# Autodesk Inventor assembly: LHSA 14
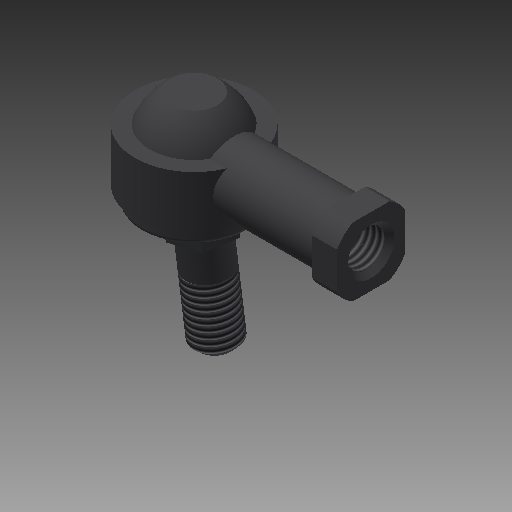
[picture p0: Inventor's stored thumbnail of the model, 512x512]
Saved by Autodesk Inventor 2018 (Build 220112000, 112)
## iProperties
Category: PARTsolutions
Company: IKO
Created: 2017-09-07
Part Number: LHSA 14
Catalog Web Link: www.cadenas.de
Description: LHSA-
Vendor: IKO
Document SubType Name: Assembly
Designer: psAdmin
Manufacturer: IKO
PSOL_IDENT_0: {$CADENAS_DATA\23d-libs\iko\iko_bearings\l_balls\lhsa_1_asmtab.prj},159 {VTYP=3D},{STYP=ASSTAB},{NB=
PSOL_IDENT_1: LHSA 14},{LINA=LHSA 14},{NN=LHSA},{DATE=13.10.2016 10:02:12},{GEOMDATE=03.01.2008},{VERSION=},{LINEI
PSOL_IDENT_2: D=90},{LINESUBID=-1},{WBVAR=}  {NB=LHSA 14},{LINA=LHSA 14},{KT=DUMMY},{IDNR=},{ORDER=LHSA 14},{RID=G
PSOL_IDENT_3: _80},{STDRT=14},{DESCR=LHSA},{TRNUMBER=},{PAST=A},{REST=O},{MASS=260},{S=M14x2},{KDM=11.546},{NDM=14
PSOL_IDENT_4: .000},{P1=2.000},{V=14},{D=38},{L=76.0},{L1=57},{L2=30},{SL1=8.0},{W=22},{W1=22},{W2=22},{D1=20.0},{
PSOL_IDENT_5: D2=25},{LL=72.0},{P=17.0},{LL1=22.5},{LL2=33.5},{LL3=22.0},{SDK=25.400},{V1=15.0},{D3=15.0000},{D4=2
PSOL_IDENT_6: 8.2138},{D5=34.0},{D6=34.00},{L3=71.2350},{L4=35.1132},{L5=38.0},{L12=39.3932},{B=12.0},{B1=7.0},{B2=
PSOL_IDENT_7: 12.0},{B3=15.0},{B4=16.8},{B5=21.8000},{LL4=8.5},{LL5=12.7},{CB=0.0},{CC=1.0},{E=0},{F=0.0},{C1=1.58
PSOL_IDENT_8: 25},{C2=2.0},{R1=5},{R2=50.6010},{R3=20.0},{R4=1.5},{CS=14600},{SS1=11.546},{S1=14},{LX=32},{LX1=36.
PSOL_IDENT_9: 6},{BL=3},{SC=1},{PPATH=lhsa_1_asmtpl.prj}
NN: LHSA
NB: LHSA 14
NBSYN: $ORDER.
LINA: LHSA 14
ORDER: LHSA 14
MASS: 260
S: M14x2
V: 14
D: 38
L: 76.0
L1: 57
L2: 30
SL1: 8.0
W1: 22
W2: 22
D1: 20.0
D2: 25
LL: 72.0
P: 17.0
LL1: 22.5
LL2: 33.5
LL3: 22.0
SDK: 25.400
CS: 14600
SUPPLIER: IKO
ARTICLENO: LHSA 14
BOMINFO: LHSA 14
CREATOR: CADENAS GmbH
Title: LHSA 14
Author: Cadenas PARTsolutions
## Documents named in this file (3)
- D:\Works\RBBR\CAD\汎用部品\エルボール14mm\LHSA 14.iam
- D:\Works\RBBR\CAD\汎用部品\エルボール14mm\LHSA 14 Body2.ipt
- D:\Works\RBBR\CAD\汎用部品\エルボール14mm\LHSA 14 Body1.ipt
## Components (2 placed, 2 different names)
1. LHSA 14 Body2:1 — ボール:1
2. LHSA 14 Body1:1 — ボール:1
## Relationships (1: BallJoint 1)
- ボール:1 [BallJoint]: LHSA 14 Body2:1 ↔ LHSA 14 Body1:1
